# Autodesk Inventor assembly: remote_assemblyv2
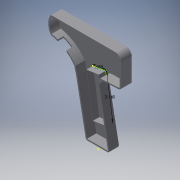
[picture p0: Inventor's stored thumbnail of the model, 180x180]
Saved by Autodesk Inventor 2019.4 (Build 234330000, 330)
## iProperties
Created: 2019-10-24
Part Number: remote_assemblyv2
Document SubType Name: Assembly
Designer: nLaptop
Author: nLaptop
## Documents named in this file (4)
- C:\Users\nLaptop\Documents\405remote housing\remote_assemblyv2.iam
- C:\Users\nLaptop\Documents\405remote housing\remote_housing_v2.ipt
- C:\Users\nLaptop\Documents\405remote housing\espHolder.ipt
- C:\Users\nLaptop\Documents\405remote housing\batteryHousing.ipt
## Components (3 placed, 3 different names)
1. remote_housing_v2:1 — Mate:2, Mate:3
2. espHolder:1 — Mate:3
3. batteryHousing:1 — Mate:2
## Relationships (2: Mate 2)
- Mate:2: remote_housing_v2:1 ↔ batteryHousing:1
- Mate:3: remote_housing_v2:1 ↔ espHolder:1
